# Autodesk Inventor assembly: COMPONENTS
(part 2 of 4)
- C:\Users\rtreacy\Documents\Inventor\SNAP Enclosure 8x10x1.75 Ver1.A\drawings\SNAP Ver2 pack-n-go\Workgroups\NotInProject\CAPC1005X50L_C306.ipt
- C:\Users\rtreacy\Documents\Inventor\SNAP Enclosure 8x10x1.75 Ver1.A\drawings\SNAP Ver2 pack-n-go\Workgroups\NotInProject\CAPC1005X50L_C311.ipt
- C:\Users\rtreacy\Documents\Inventor\SNAP Enclosure 8x10x1.75 Ver1.A\drawings\SNAP Ver2 pack-n-go\Workgroups\NotInProject\CAPC1005X50L_C287.ipt
- C:\Users\rtreacy\Documents\Inventor\SNAP Enclosure 8x10x1.75 Ver1.A\drawings\SNAP Ver2 pack-n-go\Workgroups\NotInProject\CAPC1005X50L_C309.ipt
- C:\Users\rtreacy\Documents\Inventor\SNAP Enclosure 8x10x1.75 Ver1.A\drawings\SNAP Ver2 pack-n-go\Workgroups\NotInProject\CAPC1005X50L_C3.ipt
- C:\Users\rtreacy\Documents\Inventor\SNAP Enclosure 8x10x1.75 Ver1.A\drawings\SNAP Ver2 pack-n-go\Workgroups\NotInProject\CAPC1005X50L_C42.ipt
- C:\Users\rtreacy\Documents\Inventor\SNAP Enclosure 8x10x1.75 Ver1.A\drawings\SNAP Ver2 pack-n-go\Workgroups\NotInProject\CAPC1005X50L_C81.ipt
- C:\Users\rtreacy\Documents\Inventor\SNAP Enclosure 8x10x1.75 Ver1.A\drawings\SNAP Ver2 pack-n-go\Workgroups\NotInProject\CAPC1005X50L_C45.ipt
- C:\Users\rtreacy\Documents\Inventor\SNAP Enclosure 8x10x1.75 Ver1.A\drawings\SNAP Ver2 pack-n-go\Workgroups\NotInProject\CAPC1005X50L_C6.ipt
- C:\Users\rtreacy\Documents\Inventor\SNAP Enclosure 8x10x1.75 Ver1.A\drawings\SNAP Ver2 pack-n-go\Workgroups\NotInProject\CAPC1005X50L_C84.ipt
- C:\Users\rtreacy\Documents\Inventor\SNAP Enclosure 8x10x1.75 Ver1.A\drawings\SNAP Ver2 pack-n-go\Workgroups\NotInProject\CAPC1005X50L_C12.ipt
- C:\Users\rtreacy\Documents\Inventor\SNAP Enclosure 8x10x1.75 Ver1.A\drawings\SNAP Ver2 pack-n-go\Workgroups\NotInProject\CAPC1005X50L_C181.ipt
- C:\Users\rtreacy\Documents\Inventor\SNAP Enclosure 8x10x1.75 Ver1.A\drawings\SNAP Ver2 pack-n-go\Workgroups\NotInProject\CAPC1005X50L_C139.ipt
- C:\Users\rtreacy\Documents\Inventor\SNAP Enclosure 8x10x1.75 Ver1.A\drawings\SNAP Ver2 pack-n-go\Workgroups\NotInProject\CAPC1005X50L_C76.ipt
- C:\Users\rtreacy\Documents\Inventor\SNAP Enclosure 8x10x1.75 Ver1.A\drawings\SNAP Ver2 pack-n-go\Workgroups\NotInProject\CAPC1005X50L_C37.ipt
- C:\Users\rtreacy\Documents\Inventor\SNAP Enclosure 8x10x1.75 Ver1.A\drawings\SNAP Ver2 pack-n-go\Workgroups\NotInProject\CAPC1005X50L_C115.ipt
- C:\Users\rtreacy\Documents\Inventor\SNAP Enclosure 8x10x1.75 Ver1.A\drawings\SNAP Ver2 pack-n-go\Workgroups\NotInProject\CAPC1005X50L_C75.ipt
- C:\Users\rtreacy\Documents\Inventor\SNAP Enclosure 8x10x1.75 Ver1.A\drawings\SNAP Ver2 pack-n-go\Workgroups\NotInProject\CAPC1005X50L_C36.ipt
- C:\Users\rtreacy\Documents\Inventor\SNAP Enclosure 8x10x1.75 Ver1.A\drawings\SNAP Ver2 pack-n-go\Workgroups\NotInProject\CAPC1005X50L_C114.ipt
- C:\Users\rtreacy\Documents\Inventor\SNAP Enclosure 8x10x1.75 Ver1.A\drawings\SNAP Ver2 pack-n-go\Workgroups\NotInProject\CAPC1005X50L_C74.ipt
- C:\Users\rtreacy\Documents\Inventor\SNAP Enclosure 8x10x1.75 Ver1.A\drawings\SNAP Ver2 pack-n-go\Workgroups\NotInProject\CAPC1005X50L_C136.ipt
- C:\Users\rtreacy\Documents\Inventor\SNAP Enclosure 8x10x1.75 Ver1.A\drawings\SNAP Ver2 pack-n-go\Workgroups\NotInProject\CAPC1005X50L_C183.ipt
- C:\Users\rtreacy\Documents\Inventor\SNAP Enclosure 8x10x1.75 Ver1.A\drawings\SNAP Ver2 pack-n-go\Workgroups\NotInProject\CAPC1005X50L_C35.ipt
- C:\Users\rtreacy\Documents\Inventor\SNAP Enclosure 8x10x1.75 Ver1.A\drawings\SNAP Ver2 pack-n-go\Workgroups\NotInProject\CAPC1005X50L_C113.ipt
- C:\Users\rtreacy\Documents\Inventor\SNAP Enclosure 8x10x1.75 Ver1.A\drawings\SNAP Ver2 pack-n-go\Workgroups\NotInProject\CAPC1005X50L_C175.ipt
- C:\Users\rtreacy\Documents\Inventor\SNAP Enclosure 8x10x1.75 Ver1.A\drawings\SNAP Ver2 pack-n-go\Workgroups\NotInProject\CAPC1005X50L_C174.ipt
- C:\Users\rtreacy\Documents\Inventor\SNAP Enclosure 8x10x1.75 Ver1.A\drawings\SNAP Ver2 pack-n-go\Workgroups\NotInProject\CAPC1005X50L_C171.ipt
- C:\Users\rtreacy\Documents\Inventor\SNAP Enclosure 8x10x1.75 Ver1.A\drawings\SNAP Ver2 pack-n-go\Workgroups\NotInProject\CAPC1005X50L_C166.ipt
- C:\Users\rtreacy\Documents\Inventor\SNAP Enclosure 8x10x1.75 Ver1.A\drawings\SNAP Ver2 pack-n-go\Workgroups\NotInProject\CAPC1005X50L_C165.ipt
- C:\Users\rtreacy\Documents\Inventor\SNAP Enclosure 8x10x1.75 Ver1.A\drawings\SNAP Ver2 pack-n-go\Workgroups\NotInProject\CAPC1005X50L_C185.ipt
- C:\Users\rtreacy\Documents\Inventor\SNAP Enclosure 8x10x1.75 Ver1.A\drawings\SNAP Ver2 pack-n-go\Workgroups\NotInProject\CAPC1005X50L_C163.ipt
- C:\Users\rtreacy\Documents\Inventor\SNAP Enclosure 8x10x1.75 Ver1.A\drawings\SNAP Ver2 pack-n-go\Workgroups\NotInProject\CAPC1005X50L_C72.ipt
- C:\Users\rtreacy\Documents\Inventor\SNAP Enclosure 8x10x1.75 Ver1.A\drawings\SNAP Ver2 pack-n-go\Workgroups\NotInProject\CAPC1005X50L_C135.ipt
- C:\Users\rtreacy\Documents\Inventor\SNAP Enclosure 8x10x1.75 Ver1.A\drawings\SNAP Ver2 pack-n-go\Workgroups\NotInProject\CAPC1005X50L_C131.ipt
- C:\Users\rtreacy\Documents\Inventor\SNAP Enclosure 8x10x1.75 Ver1.A\drawings\SNAP Ver2 pack-n-go\Workgroups\NotInProject\CAPC1005X50L_C129.ipt
- C:\Users\rtreacy\Documents\Inventor\SNAP Enclosure 8x10x1.75 Ver1.A\drawings\SNAP Ver2 pack-n-go\Workgroups\NotInProject\CAPC1005X50L_C127.ipt
- C:\Users\rtreacy\Documents\Inventor\SNAP Enclosure 8x10x1.75 Ver1.A\drawings\SNAP Ver2 pack-n-go\Workgroups\NotInProject\CAPC1005X50L_C123.ipt
- C:\Users\rtreacy\Documents\Inventor\SNAP Enclosure 8x10x1.75 Ver1.A\drawings\SNAP Ver2 pack-n-go\Workgroups\NotInProject\CAPC1005X50L_C33.ipt
- C:\Users\rtreacy\Documents\Inventor\SNAP Enclosure 8x10x1.75 Ver1.A\drawings\SNAP Ver2 pack-n-go\Workgroups\NotInProject\CAPC1005X50L_C111.ipt
- C:\Users\rtreacy\Documents\Inventor\SNAP Enclosure 8x10x1.75 Ver1.A\drawings\SNAP Ver2 pack-n-go\Workgroups\NotInProject\CAPC1005X50L_C89.ipt
- C:\Users\rtreacy\Documents\Inventor\SNAP Enclosure 8x10x1.75 Ver1.A\drawings\SNAP Ver2 pack-n-go\Workgroups\NotInProject\CAPC1005X50L_C50.ipt
- C:\Users\rtreacy\Documents\Inventor\SNAP Enclosure 8x10x1.75 Ver1.A\drawings\SNAP Ver2 pack-n-go\Workgroups\NotInProject\CAPC1005X50L_C11.ipt
- C:\Users\rtreacy\Documents\Inventor\SNAP Enclosure 8x10x1.75 Ver1.A\drawings\SNAP Ver2 pack-n-go\Workgroups\NotInProject\CAPC1005X50L_C70.ipt
- C:\Users\rtreacy\Documents\Inventor\SNAP Enclosure 8x10x1.75 Ver1.A\drawings\SNAP Ver2 pack-n-go\Workgroups\NotInProject\CAPC1005X50L_C31.ipt
- C:\Users\rtreacy\Documents\Inventor\SNAP Enclosure 8x10x1.75 Ver1.A\drawings\SNAP Ver2 pack-n-go\Workgroups\NotInProject\CAPC1005X50L_C109.ipt
- C:\Users\rtreacy\Documents\Inventor\SNAP Enclosure 8x10x1.75 Ver1.A\drawings\SNAP Ver2 pack-n-go\Workgroups\NotInProject\CAPC1005X50L_C69.ipt
- C:\Users\rtreacy\Documents\Inventor\SNAP Enclosure 8x10x1.75 Ver1.A\drawings\SNAP Ver2 pack-n-go\Workgroups\NotInProject\CAPC1005X50L_C30.ipt
- C:\Users\rtreacy\Documents\Inventor\SNAP Enclosure 8x10x1.75 Ver1.A\drawings\SNAP Ver2 pack-n-go\Workgroups\NotInProject\CAPC1005X50L_C121.ipt
- C:\Users\rtreacy\Documents\Inventor\SNAP Enclosure 8x10x1.75 Ver1.A\drawings\SNAP Ver2 pack-n-go\Workgroups\NotInProject\CAPC1005X50L_C119.ipt
- C:\Users\rtreacy\Documents\Inventor\SNAP Enclosure 8x10x1.75 Ver1.A\drawings\SNAP Ver2 pack-n-go\Workgroups\NotInProject\CAPC1005X50L_C108.ipt
- C:\Users\rtreacy\Documents\Inventor\SNAP Enclosure 8x10x1.75 Ver1.A\drawings\SNAP Ver2 pack-n-go\Workgroups\NotInProject\CAPC1005X50L_C78.ipt
- C:\Users\rtreacy\Documents\Inventor\SNAP Enclosure 8x10x1.75 Ver1.A\drawings\SNAP Ver2 pack-n-go\Workgroups\NotInProject\CAPC1005X50L_C39.ipt
- C:\Users\rtreacy\Documents\Inventor\SNAP Enclosure 8x10x1.75 Ver1.A\drawings\SNAP Ver2 pack-n-go\Workgroups\NotInProject\CAPC1005X50L_C117.ipt
- C:\Users\rtreacy\Documents\Inventor\SNAP Enclosure 8x10x1.75 Ver1.A\drawings\SNAP Ver2 pack-n-go\Workgroups\NotInProject\CAPC1005X50L_C104.ipt
- C:\Users\rtreacy\Documents\Inventor\SNAP Enclosure 8x10x1.75 Ver1.A\drawings\SNAP Ver2 pack-n-go\Workgroups\NotInProject\CAPC1005X50L_C64.ipt
- C:\Users\rtreacy\Documents\Inventor\SNAP Enclosure 8x10x1.75 Ver1.A\drawings\SNAP Ver2 pack-n-go\Workgroups\NotInProject\CAPC1005X50L_C1.ipt
- C:\Users\rtreacy\Documents\Inventor\SNAP Enclosure 8x10x1.75 Ver1.A\drawings\SNAP Ver2 pack-n-go\Workgroups\NotInProject\CAPC1005X50L_C40.ipt
- C:\Users\rtreacy\Documents\Inventor\SNAP Enclosure 8x10x1.75 Ver1.A\drawings\SNAP Ver2 pack-n-go\Workgroups\NotInProject\CAPC1005X50L_C79.ipt
- C:\Users\rtreacy\Documents\Inventor\SNAP Enclosure 8x10x1.75 Ver1.A\drawings\SNAP Ver2 pack-n-go\Workgroups\NotInProject\CAPC1005X50L_C10.ipt
- C:\Users\rtreacy\Documents\Inventor\SNAP Enclosure 8x10x1.75 Ver1.A\drawings\SNAP Ver2 pack-n-go\Workgroups\NotInProject\CAPC1005X50L_C49.ipt
- C:\Users\rtreacy\Documents\Inventor\SNAP Enclosure 8x10x1.75 Ver1.A\drawings\SNAP Ver2 pack-n-go\Workgroups\NotInProject\CAPC1005X50L_C88.ipt
- C:\Users\rtreacy\Documents\Inventor\SNAP Enclosure 8x10x1.75 Ver1.A\drawings\SNAP Ver2 pack-n-go\Workgroups\NotInProject\CAPC1005X50L_C67.ipt
- C:\Users\rtreacy\Documents\Inventor\SNAP Enclosure 8x10x1.75 Ver1.A\drawings\SNAP Ver2 pack-n-go\Workgroups\NotInProject\CAPC1005X50L_C28.ipt
- C:\Users\rtreacy\Documents\Inventor\SNAP Enclosure 8x10x1.75 Ver1.A\drawings\SNAP Ver2 pack-n-go\Workgroups\NotInProject\CAPC1005X50L_C106.ipt
- C:\Users\rtreacy\Documents\Inventor\SNAP Enclosure 8x10x1.75 Ver1.A\drawings\SNAP Ver2 pack-n-go\Workgroups\NotInProject\CAPC1005X50L_C66.ipt
- C:\Users\rtreacy\Documents\Inventor\SNAP Enclosure 8x10x1.75 Ver1.A\drawings\SNAP Ver2 pack-n-go\Workgroups\NotInProject\CAPC1005X50L_C27.ipt
- C:\Users\rtreacy\Documents\Inventor\SNAP Enclosure 8x10x1.75 Ver1.A\drawings\SNAP Ver2 pack-n-go\Workgroups\NotInProject\CAPC1005X50L_C105.ipt
- C:\Users\rtreacy\Documents\Inventor\SNAP Enclosure 8x10x1.75 Ver1.A\drawings\SNAP Ver2 pack-n-go\Workgroups\NotInProject\CAPC1005X50L_C65.ipt
- C:\Users\rtreacy\Documents\Inventor\SNAP Enclosure 8x10x1.75 Ver1.A\drawings\SNAP Ver2 pack-n-go\Workgroups\NotInProject\CAPC1005X50L_C26.ipt
- C:\Users\rtreacy\Documents\Inventor\SNAP Enclosure 8x10x1.75 Ver1.A\drawings\SNAP Ver2 pack-n-go\Workgroups\NotInProject\CAPC1005X50L_C25.ipt
- C:\Users\rtreacy\Documents\Inventor\SNAP Enclosure 8x10x1.75 Ver1.A\drawings\SNAP Ver2 pack-n-go\Workgroups\NotInProject\CAPC1005X50L_C102.ipt
- C:\Users\rtreacy\Documents\Inventor\SNAP Enclosure 8x10x1.75 Ver1.A\drawings\SNAP Ver2 pack-n-go\Workgroups\NotInProject\CAPC1005X50L_C103.ipt
- C:\Users\rtreacy\Documents\Inventor\SNAP Enclosure 8x10x1.75 Ver1.A\drawings\SNAP Ver2 pack-n-go\Workgroups\NotInProject\CAPC1005X50L_C63.ipt
- C:\Users\rtreacy\Documents\Inventor\SNAP Enclosure 8x10x1.75 Ver1.A\drawings\SNAP Ver2 pack-n-go\Workgroups\NotInProject\CAPC1005X50L_C24.ipt
- C:\Users\rtreacy\Documents\Inventor\SNAP Enclosure 8x10x1.75 Ver1.A\drawings\SNAP Ver2 pack-n-go\Workgroups\NotInProject\CAPC1005X50L_C61.ipt
- C:\Users\rtreacy\Documents\Inventor\SNAP Enclosure 8x10x1.75 Ver1.A\drawings\SNAP Ver2 pack-n-go\Workgroups\NotInProject\CAPC1005X50L_C100.ipt
- C:\Users\rtreacy\Documents\Inventor\SNAP Enclosure 8x10x1.75 Ver1.A\drawings\SNAP Ver2 pack-n-go\Workgroups\NotInProject\CAPC1005X50L_C22.ipt
- C:\Users\rtreacy\Documents\Inventor\SNAP Enclosure 8x10x1.75 Ver1.A\drawings\SNAP Ver2 pack-n-go\Workgroups\NotInProject\CAPC1005X50L_C601.ipt
- C:\Users\rtreacy\Documents\Inventor\SNAP Enclosure 8x10x1.75 Ver1.A\drawings\SNAP Ver2 pack-n-go\Workgroups\NotInProject\CAPC1005X50L_C602.ipt
- C:\Users\rtreacy\Documents\Inventor\SNAP Enclosure 8x10x1.75 Ver1.A\drawings\SNAP Ver2 pack-n-go\Workgroups\NotInProject\CAPC1608X90N_C120.ipt
- C:\Users\rtreacy\Documents\Inventor\SNAP Enclosure 8x10x1.75 Ver1.A\drawings\SNAP Ver2 pack-n-go\Workgroups\NotInProject\CAPC1608X90N_C124.ipt
- C:\Users\rtreacy\Documents\Inventor\SNAP Enclosure 8x10x1.75 Ver1.A\drawings\SNAP Ver2 pack-n-go\Workgroups\NotInProject\CAPC1608X90N_C128.ipt
- C:\Users\rtreacy\Documents\Inventor\SNAP Enclosure 8x10x1.75 Ver1.A\drawings\SNAP Ver2 pack-n-go\Workgroups\NotInProject\CAPC1608X90N_C132.ipt
- C:\Users\rtreacy\Documents\Inventor\SNAP Enclosure 8x10x1.75 Ver1.A\drawings\SNAP Ver2 pack-n-go\Workgroups\NotInProject\CAPC1608X90N_C179.ipt
- C:\Users\rtreacy\Documents\Inventor\SNAP Enclosure 8x10x1.75 Ver1.A\drawings\SNAP Ver2 pack-n-go\Workgroups\NotInProject\CAPC1608X90N_C150.ipt
- C:\Users\rtreacy\Documents\Inventor\SNAP Enclosure 8x10x1.75 Ver1.A\drawings\SNAP Ver2 pack-n-go\Workgroups\NotInProject\CAPC1608X90N_C140.ipt
- C:\Users\rtreacy\Documents\Inventor\SNAP Enclosure 8x10x1.75 Ver1.A\drawings\SNAP Ver2 pack-n-go\Workgroups\NotInProject\CAPC1608X90N_C161.ipt
- C:\Users\rtreacy\Documents\Inventor\SNAP Enclosure 8x10x1.75 Ver1.A\drawings\SNAP Ver2 pack-n-go\Workgroups\NotInProject\CAPC1608X90N_C169.ipt
- C:\Users\rtreacy\Documents\Inventor\SNAP Enclosure 8x10x1.75 Ver1.A\drawings\SNAP Ver2 pack-n-go\Workgroups\NotInProject\CAPC1608X90N_C190.ipt
- C:\Users\rtreacy\Documents\Inventor\SNAP Enclosure 8x10x1.75 Ver1.A\drawings\SNAP Ver2 pack-n-go\Workgroups\NotInProject\CAPC1608X90N_C218.ipt
- C:\Users\rtreacy\Documents\Inventor\SNAP Enclosure 8x10x1.75 Ver1.A\drawings\SNAP Ver2 pack-n-go\Workgroups\NotInProject\CAPC1608X90N_C221.ipt
- C:\Users\rtreacy\Documents\Inventor\SNAP Enclosure 8x10x1.75 Ver1.A\drawings\SNAP Ver2 pack-n-go\Workgroups\NotInProject\CAPC1608X90N_C229.ipt
- C:\Users\rtreacy\Documents\Inventor\SNAP Enclosure 8x10x1.75 Ver1.A\drawings\SNAP Ver2 pack-n-go\Workgroups\NotInProject\CAPC1608X90N_C236.ipt
- C:\Users\rtreacy\Documents\Inventor\SNAP Enclosure 8x10x1.75 Ver1.A\drawings\SNAP Ver2 pack-n-go\Workgroups\NotInProject\CAPC1608X90N_C243.ipt
- C:\Users\rtreacy\Documents\Inventor\SNAP Enclosure 8x10x1.75 Ver1.A\drawings\SNAP Ver2 pack-n-go\Workgroups\NotInProject\CAPC1608X90N_C252.ipt
- C:\Users\rtreacy\Documents\Inventor\SNAP Enclosure 8x10x1.75 Ver1.A\drawings\SNAP Ver2 pack-n-go\Workgroups\NotInProject\CAPC1608X90N_C261.ipt
- C:\Users\rtreacy\Documents\Inventor\SNAP Enclosure 8x10x1.75 Ver1.A\drawings\SNAP Ver2 pack-n-go\Workgroups\NotInProject\CAPC1608X90N_C193.ipt
- C:\Users\rtreacy\Documents\Inventor\SNAP Enclosure 8x10x1.75 Ver1.A\drawings\SNAP Ver2 pack-n-go\Workgroups\NotInProject\CAPC1608X90N_C215.ipt
- C:\Users\rtreacy\Documents\Inventor\SNAP Enclosure 8x10x1.75 Ver1.A\drawings\SNAP Ver2 pack-n-go\Workgroups\NotInProject\CAPC1608X90N_C21.ipt
- C:\Users\rtreacy\Documents\Inventor\SNAP Enclosure 8x10x1.75 Ver1.A\drawings\SNAP Ver2 pack-n-go\Workgroups\NotInProject\CAPC1608X90N_C60.ipt
- C:\Users\rtreacy\Documents\Inventor\SNAP Enclosure 8x10x1.75 Ver1.A\drawings\SNAP Ver2 pack-n-go\Workgroups\NotInProject\CAPC1608X90N_C99.ipt
- C:\Users\rtreacy\Documents\Inventor\SNAP Enclosure 8x10x1.75 Ver1.A\drawings\SNAP Ver2 pack-n-go\Workgroups\NotInProject\CAPC1608X90N_C38.ipt
- C:\Users\rtreacy\Documents\Inventor\SNAP Enclosure 8x10x1.75 Ver1.A\drawings\SNAP Ver2 pack-n-go\Workgroups\NotInProject\CAPC1608X90N_C116.ipt
- C:\Users\rtreacy\Documents\Inventor\SNAP Enclosure 8x10x1.75 Ver1.A\drawings\SNAP Ver2 pack-n-go\Workgroups\NotInProject\CAPC1608X90N_C73.ipt
- C:\Users\rtreacy\Documents\Inventor\SNAP Enclosure 8x10x1.75 Ver1.A\drawings\SNAP Ver2 pack-n-go\Workgroups\NotInProject\CAPC1608X90N_C34.ipt
- C:\Users\rtreacy\Documents\Inventor\SNAP Enclosure 8x10x1.75 Ver1.A\drawings\SNAP Ver2 pack-n-go\Workgroups\NotInProject\CAPC1608X90N_C112.ipt
- C:\Users\rtreacy\Documents\Inventor\SNAP Enclosure 8x10x1.75 Ver1.A\drawings\SNAP Ver2 pack-n-go\Workgroups\NotInProject\CAPC1608X90N_C71.ipt
- C:\Users\rtreacy\Documents\Inventor\SNAP Enclosure 8x10x1.75 Ver1.A\drawings\SNAP Ver2 pack-n-go\Workgroups\NotInProject\CAPC1608X90N_C32.ipt
- C:\Users\rtreacy\Documents\Inventor\SNAP Enclosure 8x10x1.75 Ver1.A\drawings\SNAP Ver2 pack-n-go\Workgroups\NotInProject\CAPC1608X90N_C110.ipt
- C:\Users\rtreacy\Documents\Inventor\SNAP Enclosure 8x10x1.75 Ver1.A\drawings\SNAP Ver2 pack-n-go\Workgroups\NotInProject\CAPC1608X90N_C77.ipt
- C:\Users\rtreacy\Documents\Inventor\SNAP Enclosure 8x10x1.75 Ver1.A\drawings\SNAP Ver2 pack-n-go\Workgroups\NotInProject\CAPC1608X90N_C68.ipt
- C:\Users\rtreacy\Documents\Inventor\SNAP Enclosure 8x10x1.75 Ver1.A\drawings\SNAP Ver2 pack-n-go\Workgroups\NotInProject\CAPC1608X90N_C29.ipt
- C:\Users\rtreacy\Documents\Inventor\SNAP Enclosure 8x10x1.75 Ver1.A\drawings\SNAP Ver2 pack-n-go\Workgroups\NotInProject\CAPC1608X90N_C107.ipt
- C:\Users\rtreacy\Documents\Inventor\SNAP Enclosure 8x10x1.75 Ver1.A\drawings\SNAP Ver2 pack-n-go\Workgroups\NotInProject\CAPC1608X90N_C62.ipt
- C:\Users\rtreacy\Documents\Inventor\SNAP Enclosure 8x10x1.75 Ver1.A\drawings\SNAP Ver2 pack-n-go\Workgroups\NotInProject\CAPC1608X90N_C23.ipt
- C:\Users\rtreacy\Documents\Inventor\SNAP Enclosure 8x10x1.75 Ver1.A\drawings\SNAP Ver2 pack-n-go\Workgroups\NotInProject\CAPC1608X90N_C101.ipt
- C:\Users\rtreacy\Documents\Inventor\SNAP Enclosure 8x10x1.75 Ver1.A\drawings\SNAP Ver2 pack-n-go\Workgroups\NotInProject\CAPC3216X180N_C134.ipt
- C:\Users\rtreacy\Documents\Inventor\SNAP Enclosure 8x10x1.75 Ver1.A\drawings\SNAP Ver2 pack-n-go\Workgroups\NotInProject\CAPC3216X180N_C138.ipt
- C:\Users\rtreacy\Documents\Inventor\SNAP Enclosure 8x10x1.75 Ver1.A\drawings\SNAP Ver2 pack-n-go\Workgroups\NotInProject\CAPC3216X180N_C141.ipt
- C:\Users\rtreacy\Documents\Inventor\SNAP Enclosure 8x10x1.75 Ver1.A\drawings\SNAP Ver2 pack-n-go\Workgroups\NotInProject\CAPC3216X180N_C143.ipt
- C:\Users\rtreacy\Documents\Inventor\SNAP Enclosure 8x10x1.75 Ver1.A\drawings\SNAP Ver2 pack-n-go\Workgroups\NotInProject\CAPC3216X180N_C144.ipt
- C:\Users\rtreacy\Documents\Inventor\SNAP Enclosure 8x10x1.75 Ver1.A\drawings\SNAP Ver2 pack-n-go\Workgroups\NotInProject\CAPC3216X180N_C231.ipt
- C:\Users\rtreacy\Documents\Inventor\SNAP Enclosure 8x10x1.75 Ver1.A\drawings\SNAP Ver2 pack-n-go\Workgroups\NotInProject\CAPC3216X180N_C238.ipt
- C:\Users\rtreacy\Documents\Inventor\SNAP Enclosure 8x10x1.75 Ver1.A\drawings\SNAP Ver2 pack-n-go\Workgroups\NotInProject\CAPC3216X180N_C245.ipt
- C:\Users\rtreacy\Documents\Inventor\SNAP Enclosure 8x10x1.75 Ver1.A\drawings\SNAP Ver2 pack-n-go\Workgroups\NotInProject\CAPC3216X180N_C254.ipt
- C:\Users\rtreacy\Documents\Inventor\SNAP Enclosure 8x10x1.75 Ver1.A\drawings\SNAP Ver2 pack-n-go\Workgroups\NotInProject\CAPC3216X180N_C263.ipt
- C:\Users\rtreacy\Documents\Inventor\SNAP Enclosure 8x10x1.75 Ver1.A\drawings\SNAP Ver2 pack-n-go\Workgroups\NotInProject\CAPC3216X180N_C314.ipt
- C:\Users\rtreacy\Documents\Inventor\SNAP Enclosure 8x10x1.75 Ver1.A\drawings\SNAP Ver2 pack-n-go\Workgroups\NotInProject\CAPC3216X180N_C316.ipt
- C:\Users\rtreacy\Documents\Inventor\SNAP Enclosure 8x10x1.75 Ver1.A\drawings\SNAP Ver2 pack-n-go\Workgroups\NotInProject\CAPC3216X180N_C320.ipt
- C:\Users\rtreacy\Documents\Inventor\SNAP Enclosure 8x10x1.75 Ver1.A\drawings\SNAP Ver2 pack-n-go\Workgroups\NotInProject\CAPC3216X180N_C322.ipt
- C:\Users\rtreacy\Documents\Inventor\SNAP Enclosure 8x10x1.75 Ver1.A\drawings\SNAP Ver2 pack-n-go\Workgroups\NotInProject\CAPC3216X180N_C146.ipt
- C:\Users\rtreacy\Documents\Inventor\SNAP Enclosure 8x10x1.75 Ver1.A\drawings\SNAP Ver2 pack-n-go\Workgroups\NotInProject\CAPC3216X180N_C197.ipt
- C:\Users\rtreacy\Documents\Inventor\SNAP Enclosure 8x10x1.75 Ver1.A\drawings\SNAP Ver2 pack-n-go\Workgroups\NotInProject\CAPC3216X180N_C145.ipt
- C:\Users\rtreacy\Documents\Inventor\SNAP Enclosure 8x10x1.75 Ver1.A\drawings\SNAP Ver2 pack-n-go\Workgroups\NotInProject\CAPC3216X180N_C149.ipt
- C:\Users\rtreacy\Documents\Inventor\SNAP Enclosure 8x10x1.75 Ver1.A\drawings\SNAP Ver2 pack-n-go\Workgroups\NotInProject\CAPC3216X180N_C155.ipt
- C:\Users\rtreacy\Documents\Inventor\SNAP Enclosure 8x10x1.75 Ver1.A\drawings\SNAP Ver2 pack-n-go\Workgroups\NotInProject\CAPC3216X180N_C158.ipt
- C:\Users\rtreacy\Documents\Inventor\SNAP Enclosure 8x10x1.75 Ver1.A\drawings\SNAP Ver2 pack-n-go\Workgroups\NotInProject\CAPC3216X180N_C156.ipt
- C:\Users\rtreacy\Documents\Inventor\SNAP Enclosure 8x10x1.75 Ver1.A\drawings\SNAP Ver2 pack-n-go\Workgroups\NotInProject\CAPC3216X180N_C159.ipt
- C:\Users\rtreacy\Documents\Inventor\SNAP Enclosure 8x10x1.75 Ver1.A\drawings\SNAP Ver2 pack-n-go\Workgroups\NotInProject\CAPC3216X180N_C212.ipt
- C:\Users\rtreacy\Documents\Inventor\SNAP Enclosure 8x10x1.75 Ver1.A\drawings\SNAP Ver2 pack-n-go\Workgroups\NotInProject\CAPC3216X180N_C213.ipt
- C:\Users\rtreacy\Documents\Inventor\SNAP Enclosure 8x10x1.75 Ver1.A\drawings\SNAP Ver2 pack-n-go\Workgroups\NotInProject\CAPC3216X180N_C214.ipt
- C:\Users\rtreacy\Documents\Inventor\SNAP Enclosure 8x10x1.75 Ver1.A\drawings\SNAP Ver2 pack-n-go\Workgroups\NotInProject\CAPC3216X180N_C228.ipt
- C:\Users\rtreacy\Documents\Inventor\SNAP Enclosure 8x10x1.75 Ver1.A\drawings\SNAP Ver2 pack-n-go\Workgroups\NotInProject\CAPC3216X180N_C235.ipt
- C:\Users\rtreacy\Documents\Inventor\SNAP Enclosure 8x10x1.75 Ver1.A\drawings\SNAP Ver2 pack-n-go\Workgroups\NotInProject\CAPC3216X180N_C242.ipt
- C:\Users\rtreacy\Documents\Inventor\SNAP Enclosure 8x10x1.75 Ver1.A\drawings\SNAP Ver2 pack-n-go\Workgroups\NotInProject\CAPC3216X180N_C251.ipt
- C:\Users\rtreacy\Documents\Inventor\SNAP Enclosure 8x10x1.75 Ver1.A\drawings\SNAP Ver2 pack-n-go\Workgroups\NotInProject\CAPC3216X180N_C260.ipt
- C:\Users\rtreacy\Documents\Inventor\SNAP Enclosure 8x10x1.75 Ver1.A\drawings\SNAP Ver2 pack-n-go\Workgroups\NotInProject\CAPC3216X180N_C232.ipt
- C:\Users\rtreacy\Documents\Inventor\SNAP Enclosure 8x10x1.75 Ver1.A\drawings\SNAP Ver2 pack-n-go\Workgroups\NotInProject\CAPC3216X180N_C239.ipt
- C:\Users\rtreacy\Documents\Inventor\SNAP Enclosure 8x10x1.75 Ver1.A\drawings\SNAP Ver2 pack-n-go\Workgroups\NotInProject\CAPC3216X180N_C246.ipt
- C:\Users\rtreacy\Documents\Inventor\SNAP Enclosure 8x10x1.75 Ver1.A\drawings\SNAP Ver2 pack-n-go\Workgroups\NotInProject\CAPC3216X180N_C255.ipt
- C:\Users\rtreacy\Documents\Inventor\SNAP Enclosure 8x10x1.75 Ver1.A\drawings\SNAP Ver2 pack-n-go\Workgroups\NotInProject\CAPC3216X180N_C264.ipt
- C:\Users\rtreacy\Documents\Inventor\SNAP Enclosure 8x10x1.75 Ver1.A\drawings\SNAP Ver2 pack-n-go\Workgroups\NotInProject\CAPC3216X180N_C248.ipt
- C:\Users\rtreacy\Documents\Inventor\SNAP Enclosure 8x10x1.75 Ver1.A\drawings\SNAP Ver2 pack-n-go\Workgroups\NotInProject\CAPC3216X180N_C257.ipt
- C:\Users\rtreacy\Documents\Inventor\SNAP Enclosure 8x10x1.75 Ver1.A\drawings\SNAP Ver2 pack-n-go\Workgroups\NotInProject\CAPC3216X180N_C266.ipt
- C:\Users\rtreacy\Documents\Inventor\SNAP Enclosure 8x10x1.75 Ver1.A\drawings\SNAP Ver2 pack-n-go\Workgroups\NotInProject\CAPC3216X180N_C268.ipt
- C:\Users\rtreacy\Documents\Inventor\SNAP Enclosure 8x10x1.75 Ver1.A\drawings\SNAP Ver2 pack-n-go\Workgroups\NotInProject\CAPC3216X180N_C290.ipt
- C:\Users\rtreacy\Documents\Inventor\SNAP Enclosure 8x10x1.75 Ver1.A\drawings\SNAP Ver2 pack-n-go\Workgroups\NotInProject\CAPMP7343X310N-ALT1_C137.ipt
- C:\Users\rtreacy\Documents\Inventor\SNAP Enclosure 8x10x1.75 Ver1.A\drawings\SNAP Ver2 pack-n-go\Workgroups\NotInProject\CAPMP7343X310N-ALT1_C233.ipt
- C:\Users\rtreacy\Documents\Inventor\SNAP Enclosure 8x10x1.75 Ver1.A\drawings\SNAP Ver2 pack-n-go\Workgroups\NotInProject\CAPMP7343X310N-ALT1_C240.ipt
- C:\Users\rtreacy\Documents\Inventor\SNAP Enclosure 8x10x1.75 Ver1.A\drawings\SNAP Ver2 pack-n-go\Workgroups\NotInProject\CAPMP7343X310N-ALT1_C247.ipt
- C:\Users\rtreacy\Documents\Inventor\SNAP Enclosure 8x10x1.75 Ver1.A\drawings\SNAP Ver2 pack-n-go\Workgroups\NotInProject\CAPMP7343X310N-ALT1_C249.ipt
- C:\Users\rtreacy\Documents\Inventor\SNAP Enclosure 8x10x1.75 Ver1.A\drawings\SNAP Ver2 pack-n-go\Workgroups\NotInProject\CAPMP7343X310N-ALT1_C256.ipt
- C:\Users\rtreacy\Documents\Inventor\SNAP Enclosure 8x10x1.75 Ver1.A\drawings\SNAP Ver2 pack-n-go\Workgroups\NotInProject\CAPMP7343X310N-ALT1_C258.ipt
- C:\Users\rtreacy\Documents\Inventor\SNAP Enclosure 8x10x1.75 Ver1.A\drawings\SNAP Ver2 pack-n-go\Workgroups\NotInProject\CAPMP7343X310N-ALT1_C265.ipt
- C:\Users\rtreacy\Documents\Inventor\SNAP Enclosure 8x10x1.75 Ver1.A\drawings\SNAP Ver2 pack-n-go\Workgroups\NotInProject\CAPMP7343X310N-ALT1_C267.ipt
- C:\Users\rtreacy\Documents\Inventor\SNAP Enclosure 8x10x1.75 Ver1.A\drawings\SNAP Ver2 pack-n-go\Workgroups\NotInProject\CAPC3225X270N_C414.ipt
- C:\Users\rtreacy\Documents\Inventor\SNAP Enclosure 8x10x1.75 Ver1.A\drawings\SNAP Ver2 pack-n-go\Workgroups\NotInProject\CAPC3225X270N_C142.ipt
- C:\Users\rtreacy\Documents\Inventor\SNAP Enclosure 8x10x1.75 Ver1.A\drawings\SNAP Ver2 pack-n-go\Workgroups\NotInProject\CAPC3225X270N_C147.ipt
- C:\Users\rtreacy\Documents\Inventor\SNAP Enclosure 8x10x1.75 Ver1.A\drawings\SNAP Ver2 pack-n-go\Workgroups\NotInProject\CAPC3225X270N_C198.ipt
- C:\Users\rtreacy\Documents\Inventor\SNAP Enclosure 8x10x1.75 Ver1.A\drawings\SNAP Ver2 pack-n-go\Workgroups\NotInProject\CAPC3225X270N_C199.ipt
- C:\Users\rtreacy\Documents\Inventor\SNAP Enclosure 8x10x1.75 Ver1.A\drawings\SNAP Ver2 pack-n-go\Workgroups\NotInProject\CAPC3225X270N_C200.ipt
- C:\Users\rtreacy\Documents\Inventor\SNAP Enclosure 8x10x1.75 Ver1.A\drawings\SNAP Ver2 pack-n-go\Workgroups\NotInProject\CAPC3225X270N_C201.ipt
- C:\Users\rtreacy\Documents\Inventor\SNAP Enclosure 8x10x1.75 Ver1.A\drawings\SNAP Ver2 pack-n-go\Workgroups\NotInProject\CAPC3225X270N_C202.ipt
- C:\Users\rtreacy\Documents\Inventor\SNAP Enclosure 8x10x1.75 Ver1.A\drawings\SNAP Ver2 pack-n-go\Workgroups\NotInProject\CAPC3225X270N_C203.ipt
- C:\Users\rtreacy\Documents\Inventor\SNAP Enclosure 8x10x1.75 Ver1.A\drawings\SNAP Ver2 pack-n-go\Workgroups\NotInProject\CAPC3225X270N_C204.ipt
- C:\Users\rtreacy\Documents\Inventor\SNAP Enclosure 8x10x1.75 Ver1.A\drawings\SNAP Ver2 pack-n-go\Workgroups\NotInProject\CAPC3225X270N_C205.ipt
- C:\Users\rtreacy\Documents\Inventor\SNAP Enclosure 8x10x1.75 Ver1.A\drawings\SNAP Ver2 pack-n-go\Workgroups\NotInProject\CAPC3225X270N_C208.ipt
- C:\Users\rtreacy\Documents\Inventor\SNAP Enclosure 8x10x1.75 Ver1.A\drawings\SNAP Ver2 pack-n-go\Workgroups\NotInProject\CAPC2012X105N_C162.ipt
- C:\Users\rtreacy\Documents\Inventor\SNAP Enclosure 8x10x1.75 Ver1.A\drawings\SNAP Ver2 pack-n-go\Workgroups\NotInProject\CAPC1005X50N_C170.ipt
- C:\Users\rtreacy\Documents\Inventor\SNAP Enclosure 8x10x1.75 Ver1.A\drawings\SNAP Ver2 pack-n-go\Workgroups\NotInProject\CAPAE830X1050D995DD305L335N_C191.ipt
- C:\Users\rtreacy\Documents\Inventor\SNAP Enclosure 8x10x1.75 Ver1.A\drawings\SNAP Ver2 pack-n-go\Workgroups\NotInProject\CAPAE830X1050D995DD305L335N_C230.ipt
- C:\Users\rtreacy\Documents\Inventor\SNAP Enclosure 8x10x1.75 Ver1.A\drawings\SNAP Ver2 pack-n-go\Workgroups\NotInProject\CAPAE830X1050D995DD305L335N_C237.ipt
- C:\Users\rtreacy\Documents\Inventor\SNAP Enclosure 8x10x1.75 Ver1.A\drawings\SNAP Ver2 pack-n-go\Workgroups\NotInProject\CAPAE830X1050D995DD305L335N_C244.ipt
- C:\Users\rtreacy\Documents\Inventor\SNAP Enclosure 8x10x1.75 Ver1.A\drawings\SNAP Ver2 pack-n-go\Workgroups\NotInProject\CAPAE830X1050D995DD305L335N_C253.ipt
- C:\Users\rtreacy\Documents\Inventor\SNAP Enclosure 8x10x1.75 Ver1.A\drawings\SNAP Ver2 pack-n-go\Workgroups\NotInProject\CAPAE830X1050D995DD305L335N_C262.ipt
- C:\Users\rtreacy\Documents\Inventor\SNAP Enclosure 8x10x1.75 Ver1.A\drawings\SNAP Ver2 pack-n-go\Workgroups\NotInProject\CAPMP7343X180N-ALT1_C402.ipt
- C:\Users\rtreacy\Documents\Inventor\SNAP Enclosure 8x10x1.75 Ver1.A\drawings\SNAP Ver2 pack-n-go\Workgroups\NotInProject\CAPMP7343X180N-ALT1_C413.ipt
- C:\Users\rtreacy\Documents\Inventor\SNAP Enclosure 8x10x1.75 Ver1.A\drawings\SNAP Ver2 pack-n-go\Workgroups\NotInProject\CAPMP7343X180N-ALT1_C400.ipt
- C:\Users\rtreacy\Documents\Inventor\SNAP Enclosure 8x10x1.75 Ver1.A\drawings\SNAP Ver2 pack-n-go\Workgroups\NotInProject\CAPMP7343X180N-ALT1_C401.ipt
- C:\Users\rtreacy\Documents\Inventor\SNAP Enclosure 8x10x1.75 Ver1.A\drawings\SNAP Ver2 pack-n-go\Workgroups\NotInProject\CAPMP7343X180N-ALT1_C206.ipt
- C:\Users\rtreacy\Documents\Inventor\SNAP Enclosure 8x10x1.75 Ver1.A\drawings\SNAP Ver2 pack-n-go\Workgroups\NotInProject\CAPMP7343X180N-ALT1_C207.ipt
- C:\Users\rtreacy\Documents\Inventor\SNAP Enclosure 8x10x1.75 Ver1.A\drawings\SNAP Ver2 pack-n-go\Workgroups\NotInProject\CAPC2012X140N_C419.ipt
- C:\Users\rtreacy\Documents\Inventor\SNAP Enclosure 8x10x1.75 Ver1.A\drawings\SNAP Ver2 pack-n-go\Workgroups\NotInProject\CAPC2012X140N_C420.ipt
- C:\Users\rtreacy\Documents\Inventor\SNAP Enclosure 8x10x1.75 Ver1.A\drawings\SNAP Ver2 pack-n-go\Workgroups\NotInProject\CAPC2012X140N_C410.ipt
- C:\Users\rtreacy\Documents\Inventor\SNAP Enclosure 8x10x1.75 Ver1.A\drawings\SNAP Ver2 pack-n-go\Workgroups\NotInProject\CAPC2012X140N_C418.ipt
- C:\Users\rtreacy\Documents\Inventor\SNAP Enclosure 8x10x1.75 Ver1.A\drawings\SNAP Ver2 pack-n-go\Workgroups\NotInProject\CAPC2012X140N_C417.ipt
- C:\Users\rtreacy\Documents\Inventor\SNAP Enclosure 8x10x1.75 Ver1.A\drawings\SNAP Ver2 pack-n-go\Workgroups\NotInProject\CAPC2012X140N_C416.ipt
- C:\Users\rtreacy\Documents\Inventor\SNAP Enclosure 8x10x1.75 Ver1.A\drawings\SNAP Ver2 pack-n-go\Workgroups\NotInProject\CAPC2012X140N_C415.ipt
- C:\Users\rtreacy\Documents\Inventor\SNAP Enclosure 8x10x1.75 Ver1.A\drawings\SNAP Ver2 pack-n-go\Workgroups\NotInProject\CAPC2012X140N_C412.ipt
- C:\Users\rtreacy\Documents\Inventor\SNAP Enclosure 8x10x1.75 Ver1.A\drawings\SNAP Ver2 pack-n-go\Workgroups\NotInProject\CAPC2012X140N_C411.ipt
- C:\Users\rtreacy\Documents\Inventor\SNAP Enclosure 8x10x1.75 Ver1.A\drawings\SNAP Ver2 pack-n-go\Workgroups\NotInProject\CAPC2012X140N_C408.ipt
- C:\Users\rtreacy\Documents\Inventor\SNAP Enclosure 8x10x1.75 Ver1.A\drawings\SNAP Ver2 pack-n-go\Workgroups\NotInProject\CAPC2012X140N_C409.ipt
- C:\Users\rtreacy\Documents\Inventor\SNAP Enclosure 8x10x1.75 Ver1.A\drawings\SNAP Ver2 pack-n-go\Workgroups\NotInProject\CAPC2012X140N_C404.ipt
- C:\Users\rtreacy\Documents\Inventor\SNAP Enclosure 8x10x1.75 Ver1.A\drawings\SNAP Ver2 pack-n-go\Workgroups\NotInProject\CAPC2012X140N_C407.ipt
- C:\Users\rtreacy\Documents\Inventor\SNAP Enclosure 8x10x1.75 Ver1.A\drawings\SNAP Ver2 pack-n-go\Workgroups\NotInProject\CAPC2012X140N_C406.ipt
- C:\Users\rtreacy\Documents\Inventor\SNAP Enclosure 8x10x1.75 Ver1.A\drawings\SNAP Ver2 pack-n-go\Workgroups\NotInProject\CAPC2012X140N_C405.ipt
- C:\Users\rtreacy\Documents\Inventor\SNAP Enclosure 8x10x1.75 Ver1.A\drawings\SNAP Ver2 pack-n-go\Workgroups\NotInProject\CAPC2012X140N_C403.ipt
- C:\Users\rtreacy\Documents\Inventor\SNAP Enclosure 8x10x1.75 Ver1.A\drawings\SNAP Ver2 pack-n-go\Workgroups\NotInProject\CAPC2012X140N_C209.ipt
- C:\Users\rtreacy\Documents\Inventor\SNAP Enclosure 8x10x1.75 Ver1.A\drawings\SNAP Ver2 pack-n-go\Workgroups\NotInProject\CAPC2012X140N_C210.ipt
- C:\Users\rtreacy\Documents\Inventor\SNAP Enclosure 8x10x1.75 Ver1.A\drawings\SNAP Ver2 pack-n-go\Workgroups\NotInProject\CAPC2012X140N_C211.ipt
- C:\Users\rtreacy\Documents\Inventor\SNAP Enclosure 8x10x1.75 Ver1.A\drawings\SNAP Ver2 pack-n-go\Workgroups\NotInProject\CAPC2012X140N_C272.ipt
- C:\Users\rtreacy\Documents\Inventor\SNAP Enclosure 8x10x1.75 Ver1.A\drawings\SNAP Ver2 pack-n-go\Workgroups\NotInProject\CAPC2012X140N_C274.ipt
- C:\Users\rtreacy\Documents\Inventor\SNAP Enclosure 8x10x1.75 Ver1.A\drawings\SNAP Ver2 pack-n-go\Workgroups\NotInProject\CAPC2012X140N_C294.ipt
- C:\Users\rtreacy\Documents\Inventor\SNAP Enclosure 8x10x1.75 Ver1.A\drawings\SNAP Ver2 pack-n-go\Workgroups\NotInProject\CAPC2012X140N_C296.ipt
- C:\Users\rtreacy\Documents\Inventor\SNAP Enclosure 8x10x1.75 Ver1.A\drawings\SNAP Ver2 pack-n-go\Workgroups\NotInProject\CAPC2012X140N_C133.ipt
- C:\Users\rtreacy\Documents\Inventor\SNAP Enclosure 8x10x1.75 Ver1.A\drawings\SNAP Ver2 pack-n-go\Workgroups\NotInProject\CAPC2012X140N_C130.ipt
- C:\Users\rtreacy\Documents\Inventor\SNAP Enclosure 8x10x1.75 Ver1.A\drawings\SNAP Ver2 pack-n-go\Workgroups\NotInProject\CAPC2012X140N_C126.ipt
- C:\Users\rtreacy\Documents\Inventor\SNAP Enclosure 8x10x1.75 Ver1.A\drawings\SNAP Ver2 pack-n-go\Workgroups\NotInProject\CAPC2012X140N_C125.ipt
- C:\Users\rtreacy\Documents\Inventor\SNAP Enclosure 8x10x1.75 Ver1.A\drawings\SNAP Ver2 pack-n-go\Workgroups\NotInProject\CAPC2012X140N_C122.ipt
- C:\Users\rtreacy\Documents\Inventor\SNAP Enclosure 8x10x1.75 Ver1.A\drawings\SNAP Ver2 pack-n-go\Workgroups\NotInProject\CAPC2012X140N_C118.ipt
- C:\Users\rtreacy\Documents\Inventor\SNAP Enclosure 8x10x1.75 Ver1.A\drawings\SNAP Ver2 pack-n-go\Workgroups\NotInProject\CAPC0603X30L_C278.ipt
- C:\Users\rtreacy\Documents\Inventor\SNAP Enclosure 8x10x1.75 Ver1.A\drawings\SNAP Ver2 pack-n-go\Workgroups\NotInProject\CAPC0603X30L_C281.ipt
- C:\Users\rtreacy\Documents\Inventor\SNAP Enclosure 8x10x1.75 Ver1.A\drawings\SNAP Ver2 pack-n-go\Workgroups\NotInProject\CAPC0603X30L_C283.ipt
- C:\Users\rtreacy\Documents\Inventor\SNAP Enclosure 8x10x1.75 Ver1.A\drawings\SNAP Ver2 pack-n-go\Workgroups\NotInProject\CAPC0603X30L_C288.ipt
- C:\Users\rtreacy\Documents\Inventor\SNAP Enclosure 8x10x1.75 Ver1.A\drawings\SNAP Ver2 pack-n-go\Workgroups\NotInProject\CAPC0603X30L_C300.ipt
- C:\Users\rtreacy\Documents\Inventor\SNAP Enclosure 8x10x1.75 Ver1.A\drawings\SNAP Ver2 pack-n-go\Workgroups\NotInProject\CAPC0603X30L_C303.ipt
- C:\Users\rtreacy\Documents\Inventor\SNAP Enclosure 8x10x1.75 Ver1.A\drawings\SNAP Ver2 pack-n-go\Workgroups\NotInProject\CAPC0603X30L_C305.ipt
- C:\Users\rtreacy\Documents\Inventor\SNAP Enclosure 8x10x1.75 Ver1.A\drawings\SNAP Ver2 pack-n-go\Workgroups\NotInProject\CAPC0603X30L_C310.ipt
- C:\Users\rtreacy\Documents\Inventor\SNAP Enclosure 8x10x1.75 Ver1.A\drawings\SNAP Ver2 pack-n-go\Workgroups\NotInProject\SOD3717X135_D10.ipt
- C:\Users\rtreacy\Documents\Inventor\SNAP Enclosure 8x10x1.75 Ver1.A\drawings\SNAP Ver2 pack-n-go\Workgroups\NotInProject\SOD3717X135_D9.ipt
- C:\Users\rtreacy\Documents\Inventor\SNAP Enclosure 8x10x1.75 Ver1.A\drawings\SNAP Ver2 pack-n-go\Workgroups\NotInProject\LEDM180X60X60N_DS1.ipt
- C:\Users\rtreacy\Documents\Inventor\SNAP Enclosure 8x10x1.75 Ver1.A\drawings\SNAP Ver2 pack-n-go\Workgroups\NotInProject\LEDM180X60X60N_DS10.ipt
- C:\Users\rtreacy\Documents\Inventor\SNAP Enclosure 8x10x1.75 Ver1.A\drawings\SNAP Ver2 pack-n-go\Workgroups\NotInProject\LEDM180X60X60N_DS11.ipt
- C:\Users\rtreacy\Documents\Inventor\SNAP Enclosure 8x10x1.75 Ver1.A\drawings\SNAP Ver2 pack-n-go\Workgroups\NotInProject\LEDM180X60X60N_DS4.ipt
- C:\Users\rtreacy\Documents\Inventor\SNAP Enclosure 8x10x1.75 Ver1.A\drawings\SNAP Ver2 pack-n-go\Workgroups\NotInProject\LEDM180X60X60N_DS5.ipt
- C:\Users\rtreacy\Documents\Inventor\SNAP Enclosure 8x10x1.75 Ver1.A\drawings\SNAP Ver2 pack-n-go\Workgroups\NotInProject\LEDM180X60X60N_DS7.ipt
- C:\Users\rtreacy\Documents\Inventor\SNAP Enclosure 8x10x1.75 Ver1.A\drawings\SNAP Ver2 pack-n-go\Workgroups\NotInProject\LEDM180X60X60N_DS8.ipt
- C:\Users\rtreacy\Documents\Inventor\SNAP Enclosure 8x10x1.75 Ver1.A\drawings\SNAP Ver2 pack-n-go\Workgroups\NotInProject\LEDM180X60X60N_DS9.ipt
- C:\Users\rtreacy\Documents\Inventor\SNAP Enclosure 8x10x1.75 Ver1.A\drawings\SNAP Ver2 pack-n-go\Workgroups\NotInProject\LEDM180X60X60N_DS2.ipt
- C:\Users\rtreacy\Documents\Inventor\SNAP Enclosure 8x10x1.75 Ver1.A\drawings\SNAP Ver2 pack-n-go\Workgroups\NotInProject\LEDM180X60X60N_DS3.ipt
- C:\Users\rtreacy\Documents\Inventor\SNAP Enclosure 8x10x1.75 Ver1.A\drawings\SNAP Ver2 pack-n-go\Workgroups\NotInProject\INDM4532X340N_L1.ipt
- C:\Users\rtreacy\Documents\Inventor\SNAP Enclosure 8x10x1.75 Ver1.A\drawings\SNAP Ver2 pack-n-go\Workgroups\NotInProject\INDM4532X340N_L10.ipt
- C:\Users\rtreacy\Documents\Inventor\SNAP Enclosure 8x10x1.75 Ver1.A\drawings\SNAP Ver2 pack-n-go\Workgroups\NotInProject\INDM4532X340N_L11.ipt
- C:\Users\rtreacy\Documents\Inventor\SNAP Enclosure 8x10x1.75 Ver1.A\drawings\SNAP Ver2 pack-n-go\Workgroups\NotInProject\INDM4532X340N_L12.ipt
- C:\Users\rtreacy\Documents\Inventor\SNAP Enclosure 8x10x1.75 Ver1.A\drawings\SNAP Ver2 pack-n-go\Workgroups\NotInProject\INDM4532X340N_L2.ipt
- C:\Users\rtreacy\Documents\Inventor\SNAP Enclosure 8x10x1.75 Ver1.A\drawings\SNAP Ver2 pack-n-go\Workgroups\NotInProject\INDM4532X340N_L3.ipt
- C:\Users\rtreacy\Documents\Inventor\SNAP Enclosure 8x10x1.75 Ver1.A\drawings\SNAP Ver2 pack-n-go\Workgroups\NotInProject\INDM4532X340N_L4.ipt
- C:\Users\rtreacy\Documents\Inventor\SNAP Enclosure 8x10x1.75 Ver1.A\drawings\SNAP Ver2 pack-n-go\Workgroups\NotInProject\INDM4532X340N_L5.ipt
- C:\Users\rtreacy\Documents\Inventor\SNAP Enclosure 8x10x1.75 Ver1.A\drawings\SNAP Ver2 pack-n-go\Workgroups\NotInProject\INDM4532X340N_L6.ipt
- C:\Users\rtreacy\Documents\Inventor\SNAP Enclosure 8x10x1.75 Ver1.A\drawings\SNAP Ver2 pack-n-go\Workgroups\NotInProject\INDM4532X340N_L8.ipt
- C:\Users\rtreacy\Documents\Inventor\SNAP Enclosure 8x10x1.75 Ver1.A\drawings\SNAP Ver2 pack-n-go\Workgroups\NotInProject\INDM4532X340N_L7.ipt
- C:\Users\rtreacy\Documents\Inventor\SNAP Enclosure 8x10x1.75 Ver1.A\drawings\SNAP Ver2 pack-n-go\Workgroups\NotInProject\INDM4532X340N_L9.ipt
- C:\Users\rtreacy\Documents\Inventor\SNAP Enclosure 8x10x1.75 Ver1.A\drawings\SNAP Ver2 pack-n-go\Workgroups\NotInProject\INDC2012X110N_L14.ipt
- C:\Users\rtreacy\Documents\Inventor\SNAP Enclosure 8x10x1.75 Ver1.A\drawings\SNAP Ver2 pack-n-go\Workgroups\NotInProject\INDC2012X110N_L13.ipt
- C:\Users\rtreacy\Documents\Inventor\SNAP Enclosure 8x10x1.75 Ver1.A\drawings\SNAP Ver2 pack-n-go\Workgroups\NotInProject\INDM9630X305N_L15.ipt
- C:\Users\rtreacy\Documents\Inventor\SNAP Enclosure 8x10x1.75 Ver1.A\drawings\SNAP Ver2 pack-n-go\Workgroups\NotInProject\INDM9630X305N_L16.ipt
- C:\Users\rtreacy\Documents\Inventor\SNAP Enclosure 8x10x1.75 Ver1.A\drawings\SNAP Ver2 pack-n-go\Workgroups\NotInProject\INDM9630X305N_L17.ipt
- C:\Users\rtreacy\Documents\Inventor\SNAP Enclosure 8x10x1.75 Ver1.A\drawings\SNAP Ver2 pack-n-go\Workgroups\NotInProject\INDM9630X305N_L18.ipt